# Autodesk Inventor assembly: mg996r_right_foot_frame
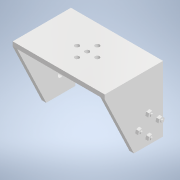
[picture p0: Inventor's stored thumbnail of the model, 180x180]
Saved by Autodesk Inventor 2021.4 (Build 254397000, 397)
## iProperties
Created: 2022-07-25
Part Number: mg996r_right_foot_frame
Document SubType Name: Assembly
Designer: isamu
Author: isamu
## Documents named in this file (5)
- D:\personal_projects\robot\inventor\2021_matlab_compat\mg996r_right_foot_frame.iam
- D:\personal_projects\robot\exports\frames\servo frame mg996 foot_MIR.ipt
- D:\personal_projects\robot\exports\handle\servo handle 4.ipt
- D:\personal_projects\robot\exports\screws\m2x8.ipt
- D:\personal_projects\robot\exports\screws\m2 nuts.ipt
## Components (10 placed, 4 different names)
1. servo frame mg996 foot_MIR:1 — Mate:1, Mate:2, Mate:3, Insert:5, Insert:6, Insert:7, Insert:8
2. servo handle 4:1 — Mate:1, Mate:2, Mate:3, Insert:1, Insert:2, Insert:3, Insert:4
3. m2x8:1 — Insert:2
4. m2x8:2 — Insert:1
5. m2x8:3 — Insert:3
6. m2x8:4 — Insert:4
7. m2 nuts:1 — Insert:8
8. m2 nuts:2 — Insert:6
9. m2 nuts:3 — Insert:5
10. m2 nuts:4 — Insert:7
## Relationships (11: Insert 8, Mate 3)
- Mate:1: servo frame mg996 foot_MIR:1 ↔ servo handle 4:1
- Mate:2: servo frame mg996 foot_MIR:1 ↔ servo handle 4:1
- Mate:3: servo frame mg996 foot_MIR:1 ↔ servo handle 4:1
- Insert:1: servo handle 4:1 ↔ m2x8:2
- Insert:2: servo handle 4:1 ↔ m2x8:1
- Insert:3: servo handle 4:1 ↔ m2x8:3
- Insert:4: servo handle 4:1 ↔ m2x8:4
- Insert:5: servo frame mg996 foot_MIR:1 ↔ m2 nuts:3
- Insert:6: servo frame mg996 foot_MIR:1 ↔ m2 nuts:2
- Insert:7: servo frame mg996 foot_MIR:1 ↔ m2 nuts:4
- Insert:8: servo frame mg996 foot_MIR:1 ↔ m2 nuts:1
